# Autodesk Inventor assembly: Bird_wing_umbralla_copy
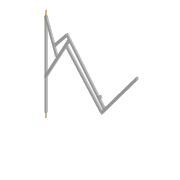
[picture p0: Inventor's stored thumbnail of the model, 180x180]
Saved by Autodesk Inventor 2022 (Build 260153000, 153)
## iProperties
Created: 2022-04-22
Part Number: Bird_wing_umbralla_copy
Document SubType Name: Assembly
Designer: dell
Author: dell
## Documents named in this file (8)
- D:\xxxx\Uni\Part IV\MECHENG_700\Part_IV_project_CAD\Bird_skeleton_prototypes\Bird_wing_umbralla_copy_V1\Bird_wing_umbralla_copy.iam
- D:\xxxx\Uni\Part IV\MECHENG_700\Part_IV_project_CAD\Bird_skeleton_prototypes\Bird_wing_umbralla_copy_V1\Part_6.ipt
- D:\xxxx\Uni\Part IV\MECHENG_700\Part_IV_project_CAD\Bird_skeleton_prototypes\Bird_wing_umbralla_copy_V1\Part_2.ipt
- D:\xxxx\Uni\Part IV\MECHENG_700\Part_IV_project_CAD\Bird_skeleton_prototypes\Bird_wing_umbralla_copy_V1\Part_3.ipt
- D:\xxxx\Uni\Part IV\MECHENG_700\Part_IV_project_CAD\Bird_skeleton_prototypes\Bird_wing_umbralla_copy_V1\Part_4.ipt
- D:\xxxx\Uni\Part IV\MECHENG_700\Part_IV_project_CAD\Bird_skeleton_prototypes\Bird_wing_umbralla_copy_V1\Part_8.ipt
- D:\xxxx\Uni\Part IV\MECHENG_700\Part_IV_project_CAD\Bird_skeleton_prototypes\Bird_wing_umbralla_copy_V1\Part_5.ipt
- D:\xxxx\Uni\Part IV\MECHENG_700\Part_IV_project_CAD\Bird_skeleton_prototypes\Bird_wing_umbralla_copy_V1\Part_7.ipt
## Components (7 placed, 7 different names)
1. Part_6:1 — Flush:2, Mate:3, Mate:4, Flush:3, Mate:11
2. Part_2:1 — Mate:4, Flush:3, Mate:5, Mate:6, Flush:4
3. Part_3:1 — Flush:2, Mate:3, Mate:5, Mate:7, Flush:5, Mate:9, Mate:11
4. Part_4:1 — Mate:6, Flush:4, Mate:8, Flush:6
5. Part_8:1 — Mate:7, Flush:5, Mate:10, Flush:7
6. Part_5:1 — Mate:8, Flush:6, Mate:9, Mate:12
7. Part_7:1 — Mate:10, Flush:7, Mate:12
## Relationships (16: Mate 10, Flush 6)
- Flush:2: Part_6:1 ↔ Part_3:1
- Mate:3: Part_6:1 ↔ Part_3:1
- Mate:4: Part_6:1 ↔ Part_2:1
- Flush:3: Part_6:1 ↔ Part_2:1
- Mate:5: Part_2:1 ↔ Part_3:1
- Mate:6: Part_2:1 ↔ Part_4:1
- Flush:4: Part_2:1 ↔ Part_4:1
- Mate:7: Part_3:1 ↔ Part_8:1
- Flush:5: Part_3:1 ↔ Part_8:1
- Mate:8: Part_4:1 ↔ Part_5:1
- Flush:6: Part_4:1 ↔ Part_5:1
- Mate:9: Part_3:1 ↔ Part_5:1
- Mate:10: Part_8:1 ↔ Part_7:1
- Flush:7: Part_8:1 ↔ Part_7:1
- Mate:11 (-100 mm): Part_6:1 ↔ Part_3:1
- Mate:12: Part_5:1 ↔ Part_7:1
